# Autodesk Inventor assembly: Lamp
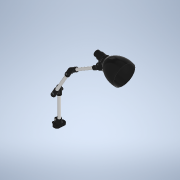
[picture p0: Inventor's stored thumbnail of the model, 180x180]
Saved by Autodesk Inventor 2020.2 (Build 242310000, 310)
## iProperties
Created: 2021-06-29
Part Number: Lamp
Document SubType Name: Assembly
Designer: JK
Author: JK
## Documents named in this file (19)
- C:\Users\JK\Documents\Inventor\Lamp\Lamp.iam
- C:\Users\JK\Documents\Inventor\Lamp\M5 washer.ipt
- C:\Users\JK\Documents\Inventor\Lamp\Aluminium tube.ipt
- C:\Users\JK\Documents\Inventor\Lamp\BallJoint.ipt
- C:\Users\JK\Documents\Inventor\Lamp\BallConnector.ipt
- C:\Users\JK\Documents\Inventor\Lamp\SocketHolder.ipt
- C:\Users\JK\Documents\Inventor\Lamp\Screen.ipt
- C:\Users\JK\Documents\Inventor\Lamp\LED Bulb.ipt
- C:\Users\JK\Documents\Inventor\Lamp\E14 socket.ipt
- C:\Users\JK\Documents\Inventor\Lamp\BallLock.ipt
- C:\Users\JK\Documents\Inventor\Lamp\M4 Nut.ipt
- C:\Users\JK\Documents\Inventor\Lamp\M4x20.ipt
- C:\Users\JK\Documents\Inventor\Lamp\ConnectorA.ipt
- C:\Users\JK\Documents\Inventor\Lamp\ConnectorB.ipt
- C:\Users\JK\Documents\Inventor\Lamp\M5 Lock nut.ipt
- C:\Users\JK\Documents\Inventor\Lamp\M5x45.ipt
- C:\Users\JK\Documents\Inventor\Lamp\M5x20.ipt
- C:\Users\JK\Documents\Inventor\Lamp\Base.ipt
- C:\Users\JK\Documents\Inventor\Lamp\M5 Nut.ipt
## Components (27 placed, 18 different names)
1. Aluminium tube:5 — Mate:36, Mate:57, Mate:58, Mate:59
2. BallConnector:1 — Mate:36, Mate:43, Mate:57
3. BallJoint:1 — Mate:40, Mate:43, Mate:49, Mate:53, Mate:56, Mate:88, Angle:9, Mate:89
4. SocketHolder:1 — Mate:40, Mate:42, Mate:47, Flush:2, Mate:53, Mate:90, Mate:91
5. Screen:1 — Mate:42, Mate:48
6. LED Bulb:1 — Mate:45, Mate:46
7. E14 socket:1 — Mate:45, Mate:46, Mate:47, Mate:48, Flush:2
8. BallLock:1 — Mate:49, Mate:50, Angle:3, Mate:51, Mate:55, Mate:56
9. M4 Nut:1 — Mate:50, Angle:3, Mate:51, Mate:54
10. M4x20:1 — Mate:54, Mate:55
11. ConnectorA:1 — Mate:58, Mate:59, Mate:60, Mate:61, Mate:62, Mate:68, Mate:69
12. ConnectorB:1 — Mate:62, Mate:63, Mate:64, Mate:65, Mate:66, Angle:4, Mate:67
13. M5 washer:1 — Mate:60, Mate:61, Mate:63
14. Aluminium tube:6 — Mate:64, Mate:65, Mate:70, Mate:71
15. M5 Lock nut:1 — Mate:66, Angle:4, Mate:67
16. M5x45:1 — Mate:68, Mate:69, Angle:7
17. ConnectorA:2 — Mate:70, Mate:71, Mate:73, Mate:75, Mate:76, Mate:81
18. ConnectorB:2 — Mate:72, Mate:73, Mate:74, Mate:77, Mate:78, Angle:5, Mate:79
19. Aluminium tube:7 — Mate:72, Mate:74, Mate:82, Mate:83
20. M5 washer:2 — Mate:75, Mate:76, Mate:77
21. M5x45:2 — Mate:80, Mate:81, Angle:6
22. M5 Lock nut:2 — Mate:78, Angle:5, Mate:79, Mate:80
23. Base:1 — Mate:82, Mate:83, Mate:84, Mate:85, Angle:8, Mate:87
24. M5x20:1 — Mate:84, Mate:85, Mate:86
25. M5 Lock nut:3 — Mate:86, Angle:8, Mate:87
26. M5 Nut:1 — Mate:88, Angle:9, Mate:89
27. M5x20:2 — Mate:90, Mate:91
## Relationships (59: Mate 50, Angle 8, Flush 1)
- Mate:36: Aluminium tube:5 ↔ BallConnector:1
- Mate:40: BallJoint:1 ↔ SocketHolder:1
- Mate:42: SocketHolder:1 ↔ Screen:1
- Mate:43: BallConnector:1 ↔ BallJoint:1
- Mate:45: LED Bulb:1 ↔ E14 socket:1
- Mate:46: LED Bulb:1 ↔ E14 socket:1
- Mate:47: SocketHolder:1 ↔ E14 socket:1
- Mate:48 (-10 mm): Screen:1 ↔ E14 socket:1
- Flush:2 (20 mm): SocketHolder:1 ↔ E14 socket:1
- Mate:49: BallJoint:1 ↔ BallLock:1
- [Angle] (0 deg): BallLock:1 ↔ M4 Nut:1
- Mate:50: BallLock:1 ↔ M4 Nut:1
- Angle:3 (0 deg): BallLock:1 ↔ M4 Nut:1
- Mate:51: BallLock:1 ↔ M4 Nut:1
- Mate:53: BallJoint:1 ↔ SocketHolder:1
- Mate:54: M4 Nut:1 ↔ M4x20:1
- Mate:55: BallLock:1 ↔ M4x20:1
- Mate:56: BallJoint:1 ↔ BallLock:1
- Mate:57: Aluminium tube:5 ↔ BallConnector:1
- Mate:58: Aluminium tube:5 ↔ ConnectorA:1
- Mate:59: Aluminium tube:5 ↔ ConnectorA:1
- Mate:60: ConnectorA:1 ↔ M5 washer:1
- Mate:61: ConnectorA:1 ↔ M5 washer:1
- Mate:62: ConnectorA:1 ↔ ConnectorB:1
- Mate:63: ConnectorB:1 ↔ M5 washer:1
- Mate:64: ConnectorB:1 ↔ Aluminium tube:6
- Mate:65: ConnectorB:1 ↔ Aluminium tube:6
- Mate:66: ConnectorB:1 ↔ M5 Lock nut:1
- Angle:4 (0 deg): ConnectorB:1 ↔ M5 Lock nut:1
- Mate:67: ConnectorB:1 ↔ M5 Lock nut:1
- Mate:68: ConnectorA:1 ↔ M5x45:1
- Mate:69: ConnectorA:1 ↔ M5x45:1
- Mate:70: Aluminium tube:6 ↔ ConnectorA:2
- Mate:71: Aluminium tube:6 ↔ ConnectorA:2
- Mate:72: ConnectorB:2 ↔ Aluminium tube:7
- Mate:73: ConnectorA:2 ↔ ConnectorB:2
- Mate:74: ConnectorB:2 ↔ Aluminium tube:7
- Mate:75: ConnectorA:2 ↔ M5 washer:2
- Mate:76: ConnectorA:2 ↔ M5 washer:2
- Mate:77: ConnectorB:2 ↔ M5 washer:2
- Mate:78: ConnectorB:2 ↔ M5 Lock nut:2
- Angle:5 (0 deg): ConnectorB:2 ↔ M5 Lock nut:2
- Mate:79: ConnectorB:2 ↔ M5 Lock nut:2
- Mate:80: M5x45:2 ↔ M5 Lock nut:2
- Mate:81: ConnectorA:2 ↔ M5x45:2
- Angle:6 (0 deg): M5x45:2
- Angle:7 (180 deg): M5x45:1
- Mate:82: Aluminium tube:7 ↔ Base:1
- Mate:83: Aluminium tube:7 ↔ Base:1
- Mate:84: Base:1 ↔ M5x20:1
- Mate:85: Base:1 ↔ M5x20:1
- Mate:86: M5x20:1 ↔ M5 Lock nut:3
- Angle:8 (0 deg): Base:1 ↔ M5 Lock nut:3
- Mate:87: Base:1 ↔ M5 Lock nut:3
- Mate:88: BallJoint:1 ↔ M5 Nut:1
- Angle:9 (0 deg): BallJoint:1 ↔ M5 Nut:1
- Mate:89: BallJoint:1 ↔ M5 Nut:1
- Mate:90: SocketHolder:1 ↔ M5x20:2
- Mate:91: SocketHolder:1 ↔ M5x20:2
